# Autodesk Inventor assembly: Ensamble terminado sin tapa y tornillos
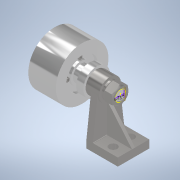
[picture p0: Inventor's stored thumbnail of the model, 180x180]
Saved by Autodesk Inventor 2021 (Build 250183000, 183)
## iProperties
Created: 2021-01-10
Part Number: Ensamble terminado sin tapa y tornillos
Document SubType Name: Assembly
Designer: dieku
Author: dieku
## Documents named in this file (5)
- C:\Users\dieku\Documents\GitHub\tallerDibujoIngenieria\Ensambles\Ensamble terminado sin tapa y tornillos.iam
- C:\Users\dieku\Documents\GitHub\tallerDibujoIngenieria\Ensambles\Ensamble eje + chaveta.iam
- C:\Users\dieku\Documents\GitHub\tallerDibujoIngenieria\Partes\anilloseparador.ipt
- C:\Users\dieku\Documents\Inventor\Content Center Files\R2021\en-US\DIN 625 - T1\DIN 625 T1 - 6304 - 20 x 52 x 15.ipt
- C:\Users\dieku\Documents\GitHub\tallerDibujoIngenieria\Partes\UNE 18035.ipt
## Components (4 placed, 4 different names)
1. Ensamble eje + chaveta:1 [sub-assembly] — Mate:1
2. anilloseparador:1 — Mate:1, Mate:3
3. DIN 625 - T1 6304 - 20 x 52 x 15:1 — Mate:2, Mate:3
4. UNE 18035:1 — Mate:2
## Relationships (3: Mate 3)
- Mate:1: Ensamble eje + chaveta:1 ↔ anilloseparador:1
- Mate:2: DIN 625 - T1 6304 - 20 x 52 x 15:1 ↔ UNE 18035:1
- Mate:3: anilloseparador:1 ↔ DIN 625 - T1 6304 - 20 x 52 x 15:1
